# Autodesk Inventor assembly: BoronProbeHead
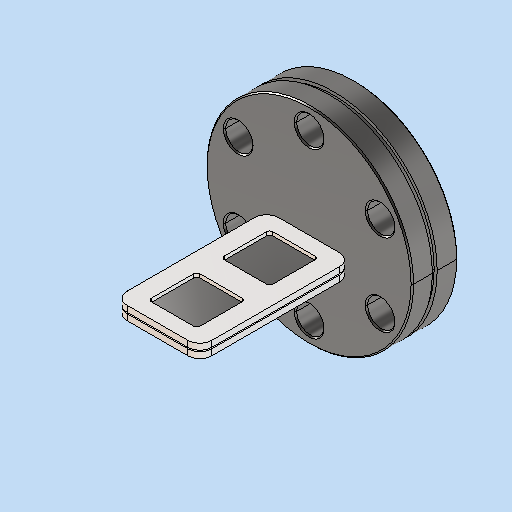
[picture p0: Inventor's stored thumbnail of the model, 512x512]
Saved by Autodesk Inventor 2025 (Build 290162000, 162)
## iProperties
Created: 2024-08-28
Part Number: BoronProbeHead
Document SubType Name: Assembly
Designer: kuzmin
Author: kuzmin
## Documents named in this file (4)
- C:\Users\queez\Dropbox\Drawings\PIHTI\BoronProbe\BoronProbeHead.iam
- C:\Users\queez\Dropbox\Drawings\PIHTI\BoronProbe\SteelSample.ipt
- C:\Users\queez\Dropbox\Drawings\PIHTI\BoronProbe\BoronProbe-flange.ipt
- C:\Users\queez\Dropbox\Drawings\PIHTI\BoronProbe\SampleTray.ipt
## Components (5 placed, 3 different names)
1. BoronProbe-flange:1 — Mate:1, Mate:2
2. SteelSample:1 — Flush:1, Flush:2, Rigid:1
3. SampleTray:1 — Mate:1, Rigid:1, Rigid:2
4. SteelSample:2 — Rigid:2, Rigid:3
5. SampleTray:2 — Mate:2, Rigid:3
## Relationships (7: WeldJoint 3, Flush 2, Mate 2)
- Flush:1 (-2 mm): SteelSample:1
- Flush:2: SteelSample:1
- Mate:1: BoronProbe-flange:1 ↔ SampleTray:1
- Rigid:1 [WeldJoint]: SteelSample:1 ↔ SampleTray:1
- Rigid:2 [WeldJoint]: SampleTray:1 ↔ SteelSample:2
- Mate:2: BoronProbe-flange:1 ↔ SampleTray:2
- Rigid:3 [WeldJoint]: SteelSample:2 ↔ SampleTray:2
